# Autodesk Inventor assembly: model_ris
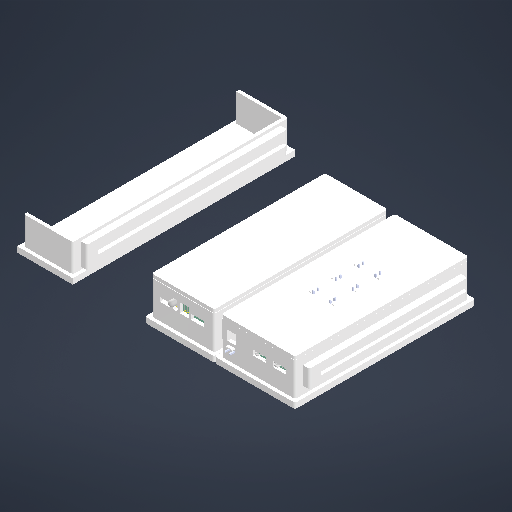
[picture p0: Inventor's stored thumbnail of the model, 512x512]
Saved by Autodesk Inventor 2025.2 (Build 292293000, 293)
## iProperties
Created: 2025-09-05
Part Number: model_ris
Document SubType Name: Assembly
Designer: sam
Author: sam
## Documents named in this file (4)
- G:\projects\primary\regulated-irrigation-system\model\asm\model_ris.iam
- G:\projects\primary\regulated-irrigation-system\model\asm\module-command\module_command.iam
- G:\projects\primary\regulated-irrigation-system\model\asm\module-switch\module_switch.iam
- G:\projects\primary\regulated-irrigation-system\model\asm\module-valve\module_valve.iam
## Components (3 placed, 3 different names)
1. module_command:1 [sub-assembly] — Mate:1, Mate:2, Mate:3
2. module_switch:1 [sub-assembly] — Mate:1, Mate:2, Mate:3
3. module_valve:1 [sub-assembly]
## Relationships (3: Mate 3)
- Mate:1: module_command:1 ↔ module_switch:1
- Mate:2 (0.2 mm): module_command:1 ↔ module_switch:1
- Mate:3 (0.2 mm): module_command:1 ↔ module_switch:1
